# Autodesk Inventor assembly: Сборка22
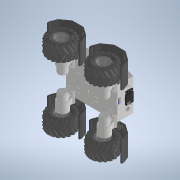
[picture p0: Inventor's stored thumbnail of the model, 180x180]
Saved by Autodesk Inventor 2022 (Build 260153000, 153)
## iProperties
Created: 2023-05-24
Part Number: Сборка22
Document SubType Name: Assembly
Designer: korsh624
Author: korsh624
## Documents named in this file (7)
- C:\git\robot_01\design\Сборка22 — копия.iam
- C:\git\robot_01\design\Сборка2.iam
- C:\git\robot_01\design\akum12v.ipt
- C:\git\robot_01\design\akkum16v.ipt
- C:\git\robot_01\design\korob\3Dkrish.ipt
- C:\git\robot_01\design\CAMERA PI COM LENTE.ipt
- C:\git\robot_01\design\goruntu modulu.ipt
## Components (6 placed, 6 different names)
1. Сборка2:1 [sub-assembly] — Совмещение:1, Совмещение:2, Совмещение:3, Заподлицо:4, Заподлицо:5, Заподлицо:6
2. akum12v:1 — Совмещение:2, Заподлицо:3, Заподлицо:5
3. akkum16v:1 — Совмещение:1, Заподлицо:3, Совмещение:3, Заподлицо:6
4. 3Dkrish:1 — Заподлицо:4, Совмещение:4, Совмещение:5
5. CAMERA PI COM LENTE:1 — Совмещение:4
6. goruntu modulu:1 — Совмещение:5
## Relationships (9: Mate 5, Flush 4)
- Совмещение:1 [Mate]: Сборка2:1 ↔ akkum16v:1
- Совмещение:2 [Mate]: Сборка2:1 ↔ akum12v:1
- Заподлицо:3 [Flush]: akum12v:1 ↔ akkum16v:1
- Совмещение:3 [Mate]: Сборка2:1 ↔ akkum16v:1
- Заподлицо:4 [Flush]: Сборка2:1 ↔ 3Dkrish:1
- Заподлицо:5 [Flush]: Сборка2:1 ↔ akum12v:1
- Заподлицо:6 [Flush]: Сборка2:1 ↔ akkum16v:1
- Совмещение:4 [Mate]: 3Dkrish:1 ↔ CAMERA PI COM LENTE:1
- Совмещение:5 [Mate]: 3Dkrish:1 ↔ goruntu modulu:1
